# Autodesk Inventor assembly: test-model-2025stp2
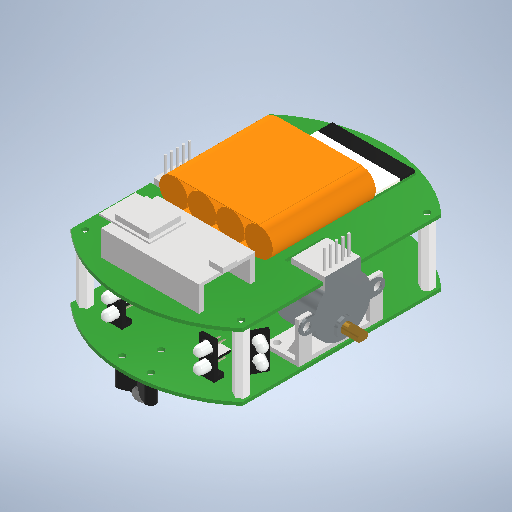
[picture p0: Inventor's stored thumbnail of the model, 512x512]
Saved by Autodesk Inventor 2025 (Build 290162000, 162)
## iProperties
Created: 2025-05-29
Part Number: test-model-2025stp2
Document SubType Name: Assembly
Designer: yamashita1
Author: yamashita1
## Documents named in this file (11)
- G:\マイドライブ\project\micro-mouse\3D-Model\test-model-2025stp2.iam
- G:\マイドライブ\project\micro-mouse\3D-Model\BaseBoard2.ipt
- G:\マイドライブ\project\micro-mouse\3D-Model\BallCaster-H16.ipt
- G:\マイドライブ\project\micro-mouse\3D-Model\Photo-Sensor.iam
- G:\マイドライブ\project\micro-mouse\3D-Model\ESP32-DevKitC.ipt
- G:\マイドライブ\project\micro-mouse\3D-Model\NiMH-Battery.ipt
- G:\マイドライブ\project\micro-mouse\3D-Model\AQM1602Y.ipt
- G:\マイドライブ\project\micro-mouse\3D-Model\D-Shaft_Wheel4.ipt
- G:\マイドライブ\project\micro-mouse\3D-Model\Stepper-28BYJ_asm.iam
- G:\マイドライブ\project\micro-mouse\3D-Model\Spacer-M3H30.ipt
- G:\マイドライブ\project\micro-mouse\3D-Model\BaseBoard3.ipt
## Components (19 placed, 10 different names)
1. BaseBoard2:1 — メイト:7, メイト:8, メイト:9, メイト:18, メイト:19, メイト:20, メイト:21, メイト:46, メイト:47, メイト:48, メイト:49, メイト:50, メイト:52, メイト:53, メイト:54, メイト:55, メイト:59, メイト:60, メイト:61, メイト:62
2. BallCaster-H16:1 — メイト:7, メイト:8, メイト:9
3. Photo-Sensor:1 [sub-assembly] — メイト:18
4. Photo-Sensor:2 [sub-assembly] — メイト:19
5. Photo-Sensor:3 [sub-assembly] — メイト:20
6. Photo-Sensor:4 [sub-assembly] — メイト:21
7. ESP32-DevKitC:1 — メイト:66
8. NiMH-Battery:1 — メイト:68
9. AQM1602Y:1 — メイト:67
10. D-Shaft_Wheel4:1
11. D-Shaft_Wheel4:2
12. BallCaster-H16:2 — メイト:46, メイト:47, メイト:48
13. Stepper-28BYJ_asm:1 [sub-assembly] — メイト:49
14. Stepper-28BYJ_asm:2 [sub-assembly] — メイト:50
15. Spacer-M3H30:1 — メイト:52, メイト:59, メイト:63
16. Spacer-M3H30:2 — メイト:53, メイト:60
17. Spacer-M3H30:3 — メイト:54, メイト:62
18. Spacer-M3H30:4 — メイト:55, メイト:61, メイト:64, メイト:65
19. BaseBoard3:1 — メイト:63, メイト:64, メイト:65, メイト:66, メイト:67, メイト:68
## Relationships (26: Mate 26)
- メイト:7 [Mate]: BaseBoard2:1 ↔ BallCaster-H16:1
- メイト:8 [Mate]: BaseBoard2:1 ↔ BallCaster-H16:1
- メイト:9 [Mate]: BaseBoard2:1 ↔ BallCaster-H16:1
- メイト:18 [Mate]: BaseBoard2:1 ↔ Photo-Sensor:1
- メイト:19 [Mate]: BaseBoard2:1 ↔ Photo-Sensor:2
- メイト:20 [Mate]: BaseBoard2:1 ↔ Photo-Sensor:3
- メイト:21 [Mate]: BaseBoard2:1 ↔ Photo-Sensor:4
- メイト:46 [Mate]: BaseBoard2:1 ↔ BallCaster-H16:2
- メイト:47 [Mate]: BaseBoard2:1 ↔ BallCaster-H16:2
- メイト:48 [Mate]: BaseBoard2:1 ↔ BallCaster-H16:2
- メイト:49 [Mate]: BaseBoard2:1 ↔ Stepper-28BYJ_asm:1
- メイト:50 [Mate]: BaseBoard2:1 ↔ Stepper-28BYJ_asm:2
- メイト:52 [Mate]: BaseBoard2:1 ↔ Spacer-M3H30:1
- メイト:53 [Mate]: BaseBoard2:1 ↔ Spacer-M3H30:2
- メイト:54 [Mate]: BaseBoard2:1 ↔ Spacer-M3H30:3
- メイト:55 [Mate]: BaseBoard2:1 ↔ Spacer-M3H30:4
- メイト:59 [Mate]: BaseBoard2:1 ↔ Spacer-M3H30:1
- メイト:60 [Mate]: BaseBoard2:1 ↔ Spacer-M3H30:2
- メイト:61 [Mate]: BaseBoard2:1 ↔ Spacer-M3H30:4
- メイト:62 [Mate]: BaseBoard2:1 ↔ Spacer-M3H30:3
- メイト:63 [Mate]: Spacer-M3H30:1 ↔ BaseBoard3:1
- メイト:64 [Mate]: Spacer-M3H30:4 ↔ BaseBoard3:1
- メイト:65 [Mate]: Spacer-M3H30:4 ↔ BaseBoard3:1
- メイト:66 [Mate]: ESP32-DevKitC:1 ↔ BaseBoard3:1
- メイト:67 [Mate]: AQM1602Y:1 ↔ BaseBoard3:1
- メイト:68 [Mate] (5 mm): NiMH-Battery:1 ↔ BaseBoard3:1
